# Autodesk Inventor assembly: CableBraider
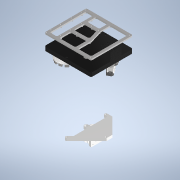
[picture p0: Inventor's stored thumbnail of the model, 180x180]
Saved by Autodesk Inventor 2022 (Build 260153000, 153)
## iProperties
Created: 2020-07-21
Part Number: CableBraider
Document SubType Name: Assembly
Designer: elmar
Author: elmar
## Documents named in this file (9)
- C:\repo\FourWireBraidingMachine\MetalCableBraider\CableBraider.iam
- C:\repo\FourWireBraidingMachine\MetalCableBraider\BasePlate.ipt
- C:\repo\FourWireBraidingMachine\MetalCableBraider\WinderAssembly.iam
- C:\Users\Eric\OneDrive\Documents\Inventor\Content Center Files\R2022\en-US\ANSI B18.2.4.2M\ANSI B18.2.4.2M - M8x1.25 - 13.ipt
- C:\repo\FourWireBraidingMachine\MetalCableBraider\Carriage.iam
- C:\repo\FourWireBraidingMachine\MetalCableBraider\NEMA17.ipt
- C:\repo\FourWireBraidingMachine\MetalCableBraider\ElectronicsPlate.ipt
- C:\repo\FourWireBraidingMachine\MetalCableBraider\DriveGearNEMA17.ipt
- C:\repo\FourWireBraidingMachine\MetalCableBraider\TwoPartHornGear.ipt
## Components (9 placed, 8 different names)
1. BasePlate:1 — Mate:1, Mate:2, Mate:3, Insert:55, Insert:62, Mate:10
2. TwoPartHornGear:1 — Angle:3, Insert:55, Flush:3
3. TwoPartHornGear:2 — Angle:3
4. WinderAssembly:1 [sub-assembly]
5. ANSI B18.2.4.2M M8x1.25:2
6. Carriage:1 [sub-assembly]
7. NEMA17:1 — Insert:62, Mate:10, Mate:12, Angle:4
8. ElectronicsPlate:1
9. DriveGearNEMA17:1 — Mate:12, Flush:3, Angle:4
## Relationships (10: Mate 5, Angle 2, Insert 2, Flush 1)
- Mate:1: BasePlate:1
- Mate:2: BasePlate:1
- Mate:3: BasePlate:1
- Angle:3 (0 deg): TwoPartHornGear:1 ↔ TwoPartHornGear:2
- Insert:55 (1 mm): BasePlate:1 ↔ TwoPartHornGear:1
- Insert:62: BasePlate:1 ↔ NEMA17:1
- Mate:10: BasePlate:1 ↔ NEMA17:1
- Mate:12: NEMA17:1 ↔ DriveGearNEMA17:1
- Flush:3: TwoPartHornGear:1 ↔ DriveGearNEMA17:1
- Angle:4 (180 deg): NEMA17:1 ↔ DriveGearNEMA17:1
